# Autodesk Inventor assembly: mgn_assy
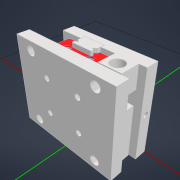
[picture p0: Inventor's stored thumbnail of the model, 180x180]
Saved by Autodesk Inventor 2022 (Build 260153000, 153)
## iProperties
Created: 2021-06-28
Part Number: mgn_assy
Document SubType Name: Assembly
Designer: user
Author: user
## Documents named in this file (6)
- Z:\_VMTransfer\_Inventor_Projects\LF_3D_Printer\Idex_Dovetail\mgn_assy.iam
- Z:\_VMTransfer\_Inventor_Projects\LF_3D_Printer\Idex_Dovetail\Master.ipt
- Z:\_VMTransfer\_Inventor_Projects\LF_3D_Printer\Idex_Dovetail\MGN_Mount.ipt
- C:\Users\user\Documents\Inventor\Content Center Files\R2022\en-US\MGN12-Rail\MGN12-50.ipt
- C:\Users\user\Documents\Inventor\Content Center Files\R2022\en-US\MGN12H_Block\MGN12H.ipt
- Z:\_VMTransfer\_Inventor_Projects\LF_3D_Printer\Idex_Dovetail\mgn_screw_nut.ipt
## Components (7 placed, 5 different names)
1. Master:1 — Insert:2, Insert:3
2. MGN_Mount:1 — Insert:1, Insert:2, Insert:3, Insert:4, Insert:7, Insert:8, Cylindrical:1
3. MGN12-50:1 — Insert:1, Mate:1, Mate:2, Insert:4
4. MGN12H:1 — Mate:1, Mate:2, Insert:5, Insert:6
5. Master:2 — Insert:5, Insert:6, Insert:9
6. MGN12H:2 — Insert:7, Insert:8
7. mgn_screw_nut:1 — Insert:9, Cylindrical:1
## Relationships (12: Insert 9, Mate 2, CylindricalJoint 1)
- Insert:1: MGN_Mount:1 ↔ MGN12-50:1
- Mate:1: MGN12-50:1 ↔ MGN12H:1
- Mate:2: MGN12-50:1 ↔ MGN12H:1
- Insert:2: Master:1 ↔ MGN_Mount:1
- Insert:3: Master:1 ↔ MGN_Mount:1
- Insert:4: MGN_Mount:1 ↔ MGN12-50:1
- Insert:5: MGN12H:1 ↔ Master:2
- Insert:6: MGN12H:1 ↔ Master:2
- Insert:7: MGN_Mount:1 ↔ MGN12H:2
- Insert:8: MGN_Mount:1 ↔ MGN12H:2
- Insert:9: Master:2 ↔ mgn_screw_nut:1
- Cylindrical:1: MGN_Mount:1 ↔ mgn_screw_nut:1
